# Autodesk Inventor assembly: motor_holder_assemble
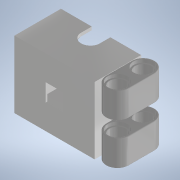
[picture p0: Inventor's stored thumbnail of the model, 180x180]
Saved by Autodesk Inventor 2021 (Build 250183000, 183)
## iProperties
Created: 2024-05-29
Part Number: motor_holder_assemble
Document SubType Name: Assembly
Designer: 23adrdam
Author: 23adrdam
## Documents named in this file (3)
- C:\Users\23adrdam\Desktop\driverbot\driverbot-adrian\models\motor_holder_assemble.iam
- C:\Users\23adrdam\Desktop\driverbot\driverbot-adrian\models\Imported Components\motor_holder#2\motor_holder#2.ipt
- C:\Users\23adrdam\Desktop\driverbot\driverbot-adrian\models\Imported Components\BEAM 2_\BEAM 2_.ipt
## Components (3 placed, 2 different names)
1. motor_holder#2:1 — Mate:1, Mate:2, Mate:3, Mate:4
2. BEAM 2_:1 — Mate:1, Mate:2, Mate:5
3. BEAM 2_:2 — Mate:3, Mate:4, Mate:5
## Relationships (5: Mate 5)
- Mate:1: motor_holder#2:1 ↔ BEAM 2_:1
- Mate:2: motor_holder#2:1 ↔ BEAM 2_:1
- Mate:3: motor_holder#2:1 ↔ BEAM 2_:2
- Mate:4: motor_holder#2:1 ↔ BEAM 2_:2
- Mate:5: BEAM 2_:1 ↔ BEAM 2_:2
